# Autodesk Inventor assembly: zloeznie
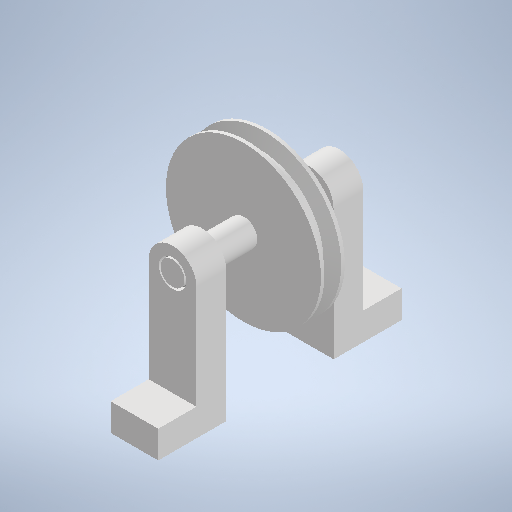
[picture p0: Inventor's stored thumbnail of the model, 512x512]
Saved by Autodesk Inventor 2025 (Build 290162000, 162)
## iProperties
Created: 2025-05-28
Part Number: zloeznie
Document SubType Name: Assembly
Designer: tjaku
Author: tjaku
## Documents named in this file (6)
- C:\Users\tjaku\OneDrive\Pulpit\zloeznie.iam
- C:\Users\tjaku\OneDrive\Pulpit\waleczek.ipt
- C:\Users\tjaku\OneDrive\Pulpit\Podstawa.ipt
- C:\Users\tjaku\Downloads\flanged_bushing_pcmf_pcmf_202321_5_e.ipt
- C:\Users\tjaku\OneDrive\Pulpit\Kolo.ipt
- C:\Users\tjaku\OneDrive\Pulpit\tuleja_dys.ipt
## Components (10 placed, 5 different names)
1. waleczek:1 — Zestawiające:7, Zestawiające:8, Zestawiające:11, Zestawiające:12, Zestawiające:13, Zestawiające:15, Zestawiające:17, Zestawiające:19
2. Podstawa:2 — Zestawiające:2, Zestawiające:4
3. Podstawa:3 — Zestawiające:5, Zestawiające:6, Zestawiające:8
4. flanged_bushing_pcmf_pcmf_202321_5_e:1 — Zestawiające:5, Zestawiające:6, Zestawiające:7, Zestawiające:16
5. flanged_bushing_pcmf_pcmf_202321_5_e:2 — Zestawiające:2, Zestawiające:4
6. Podstawa:4 — Zestawiające:9, Zestawiające:10, Zestawiające:11, Zestawiające:12, Zestawiające:13
7. flanged_bushing_pcmf_pcmf_202321_5_e:3 — Zestawiające:9, Zestawiające:10, Zestawiające:18
8. Kolo:1 — Zestawiające:19, Zestawiające:20
9. tuleja_dys:1 — Zestawiające:15, Zestawiające:16, Zestawiające:20
10. tuleja_dys:2 — Zestawiające:17, Zestawiające:18
## Relationships (17: Mate 17)
- Zestawiające:2 [Mate]: Podstawa:2 ↔ flanged_bushing_pcmf_pcmf_202321_5_e:2
- Zestawiające:4 [Mate]: Podstawa:2 ↔ flanged_bushing_pcmf_pcmf_202321_5_e:2
- Zestawiające:5 [Mate]: Podstawa:3 ↔ flanged_bushing_pcmf_pcmf_202321_5_e:1
- Zestawiające:6 [Mate]: Podstawa:3 ↔ flanged_bushing_pcmf_pcmf_202321_5_e:1
- Zestawiające:7 [Mate]: waleczek:1 ↔ flanged_bushing_pcmf_pcmf_202321_5_e:1
- Zestawiające:8 [Mate]: waleczek:1 ↔ Podstawa:3
- Zestawiające:9 [Mate]: Podstawa:4 ↔ flanged_bushing_pcmf_pcmf_202321_5_e:3
- Zestawiające:10 [Mate]: Podstawa:4 ↔ flanged_bushing_pcmf_pcmf_202321_5_e:3
- Zestawiające:11 [Mate]: waleczek:1 ↔ Podstawa:4
- Zestawiające:12 [Mate]: waleczek:1 ↔ Podstawa:4
- Zestawiające:13 [Mate]: waleczek:1 ↔ Podstawa:4
- Zestawiające:15 [Mate]: waleczek:1 ↔ tuleja_dys:1
- Zestawiające:16 [Mate]: flanged_bushing_pcmf_pcmf_202321_5_e:1 ↔ tuleja_dys:1
- Zestawiające:17 [Mate]: waleczek:1 ↔ tuleja_dys:2
- Zestawiające:18 [Mate]: flanged_bushing_pcmf_pcmf_202321_5_e:3 ↔ tuleja_dys:2
- Zestawiające:19 [Mate]: waleczek:1 ↔ Kolo:1
- Zestawiające:20 [Mate]: Kolo:1 ↔ tuleja_dys:1
